# Autodesk Inventor assembly: Case
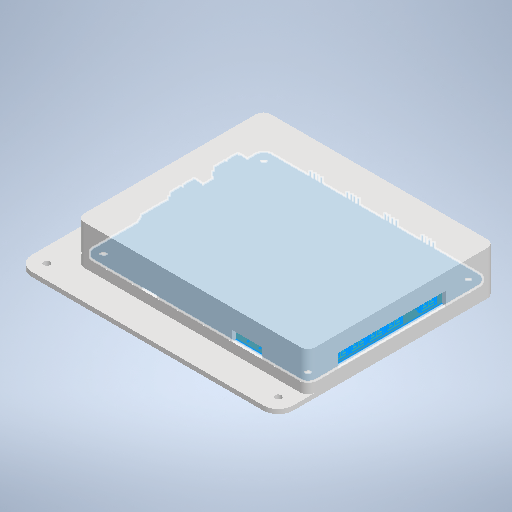
[picture p0: Inventor's stored thumbnail of the model, 512x512]
Saved by Autodesk Inventor 2025.2 (Build 292293000, 293)
## iProperties
Created: 2026-05-08
Part Number: Case
Document SubType Name: Assembly
Designer: Simon
Author: Simon
## Documents named in this file (4)
- C:\Users\Simon\Projects\BEng Mechatronics\Hydrogel-3D-Printer\Hardware\Bioprinter Machine Design\Final System\Electronics Case\Case.iam
- C:\Users\Simon\Projects\BEng Mechatronics\Hydrogel-3D-Printer\Hardware\Bioprinter Machine Design\Final System\Electronics Case\BottomCase.ipt
- C:\Users\Simon\Projects\BEng Mechatronics\Hydrogel-3D-Printer\Hardware\Bioprinter Machine Design\Final System\Electronics Case\TopCase.ipt
- C:\Users\Simon\Projects\BEng Mechatronics\Hydrogel-3D-Printer\Hardware\Bioprinter Machine Design\Final System\Electronics Case\PCB\HydrogelBioprinter.iam
## Components (3 placed, 3 different names)
1. BottomCase:1 — Mate:4, Mate:5, Mate:6, Mate:7, Mate:8
2. TopCase:1 — Mate:4, Mate:5
3. HydrogelBioprinter:1 [sub-assembly] — Mate:6, Mate:7, Mate:8
## Relationships (5: Mate 5)
- Mate:4: BottomCase:1 ↔ TopCase:1
- Mate:5: BottomCase:1 ↔ TopCase:1
- Mate:6: BottomCase:1 ↔ HydrogelBioprinter:1
- Mate:7: BottomCase:1 ↔ HydrogelBioprinter:1
- Mate:8: BottomCase:1 ↔ HydrogelBioprinter:1
